# Autodesk Inventor assembly: CL4-400-GB
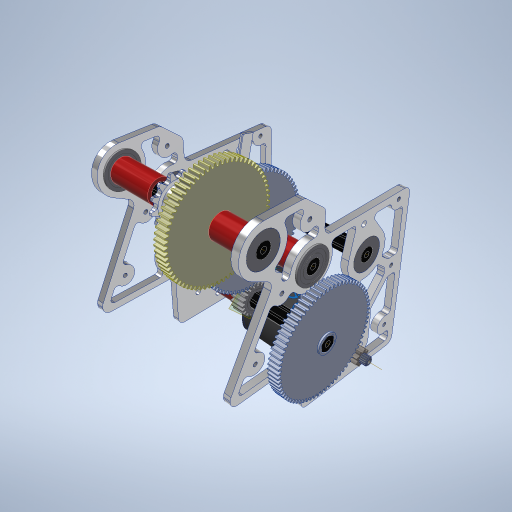
[picture p0: Inventor's stored thumbnail of the model, 512x512]
Saved by Autodesk Inventor 2023.4 (Build 274418000, 418)
## iProperties
Created: 2025-02-08
Part Number: CL4-400-GB
Document SubType Name: Assembly
Designer: slick
Mass: 1317.22 g
Surface Area: 2022.83 cm^2
Volume: 570.049 cm^3
Density: 2.31072 g/cm^3
Author: slick
## Documents named in this file (23)
- C:\Users\jmcintyr\Documents\GitHub\2025-ReefScape---CAD\Climber\CL4\CL4-400-GB.iam
- C:\Users\jmcintyr\Documents\GitHub\2025-ReefScape---CAD\Climber\CL4\CL4-016.ipt
- C:\Users\jmcintyr\Documents\GitHub\2025-ReefScape---CAD\COMMON PARTS\BEARINGS\0_500_ID_x_1_125_OD_x_0_313_WD_Flanged_Bearing_217-2731.ipt
- C:\Users\jmcintyr\Documents\GitHub\2025-ReefScape---CAD\COMMON PARTS\MOTORS\Kracken with Cover and Boards.iam
- C:\Users\jmcintyr\Documents\GitHub\2025-ReefScape---CAD\COMMON PARTS\GEARS\WCP-1006\WCP-1006.ipt
- C:\Users\jmcintyr\Documents\GitHub\2025-ReefScape---CAD\COMMON PARTS\GEARS\20dp .5 hex\72t_Aluminum_Spur_Gear_20_DP_1_2_Hex_Bore_217-3576.ipt
- C:\Users\jmcintyr\Documents\GitHub\2025-ReefScape---CAD\COMMON PARTS\GEARS\20dp .5 hex\20t_Aluminum_Spur_Gear_20_DP_1_2_Hex_Bore_217-2702.ipt
- C:\Users\jmcintyr\Documents\GitHub\2025-ReefScape---CAD\COMMON PARTS\GEARS\20dp .5 hex\68t_Aluminum_Spur_Gear_20_DP_1_2_Hex_Bore_217-5477.ipt
- C:\Users\jmcintyr\Documents\GitHub\2025-ReefScape---CAD\Climber\CL4\CL4-018.ipt
- C:\Users\jmcintyr\Documents\GitHub\2025-ReefScape---CAD\Climber\CL4\CL4-019.ipt
- C:\Users\jmcintyr\Documents\GitHub\2025-ReefScape---CAD\COMMON PARTS\BEARINGS\13_75mm_1_2_ThunderHex_ID_x_1_125_OD_x_0_313_WD_Flanged_Bearing_217-4006_MIR.ipt
- C:\Users\jmcintyr\Documents\GitHub\2025-ReefScape---CAD\Climber\CL4\CL4-020.ipt
- C:\Users\jmcintyr\Documents\GitHub\2025-ReefScape---CAD\COMMON PARTS\HUBS\WCP-1388.ipt
- C:\Users\jmcintyr\Documents\GitHub\2025-ReefScape---CAD\STEP files\5163A16_Ratcheting Combination Wrench stubby.ipt
- C:\Users\jmcintyr\Documents\GitHub\2025-ReefScape---CAD\Climber\CL4\CL4-024.ipt
- C:\Users\jmcintyr\Documents\GitHub\2025-ReefScape---CAD\Climber\CL4\CL4-025.ipt
- C:\Users\jmcintyr\Documents\GitHub\2025-ReefScape---CAD\Climber\Spacers\CL-S-001.ipt
- C:\Users\jmcintyr\Documents\GitHub\2025-ReefScape---CAD\Climber\Spacers\CL-S-002.ipt
- C:\Users\jmcintyr\Documents\GitHub\2025-ReefScape---CAD\Climber\Spacers\CL-S-003.ipt
- C:\Users\jmcintyr\Documents\GitHub\2025-ReefScape---CAD\Climber\Spacers\CL-S-005.ipt
- C:\Users\jmcintyr\Documents\GitHub\2025-ReefScape---CAD\Climber\Spacers\CL-S-007.ipt
- C:\Users\jmcintyr\Documents\GitHub\2025-ReefScape---CAD\COMMON PARTS\SPROCKETS\35\12t_Aluminum_Hub_Sprocket_35_Chain_1_2_Hex_Bore_217-2662.ipt
- C:\Users\jmcintyr\Documents\GitHub\2025-ReefScape---CAD\COMMON PARTS\MOTORS\X 60 MOTOR SPACER.ipt
## Components (36 placed, 22 different names)
1. CL4-016:1 — Mate:1, Mate:2, Mate:3, Mate:4, Symmetry:1, Mate:19, Mate:20, Insert:8, Insert:14, Insert:15, Insert:17, Insert:22
2. CL4-016:2 — Mate:1, Mate:2, Mate:3, Symmetry:1, Insert:11, Insert:12, Insert:13, Insert:16, Mate:34, Insert:18
3. 0_500_ID_x_1_125_OD_x_0_313_WD_Flanged_Bearing_217-2731:1 — Insert:12, Mate:26, Flush:6, Mate:53
4. 0_500_ID_x_1_125_OD_x_0_313_WD_Flanged_Bearing_217-2731:2 — Insert:13, Mate:23, Flush:4, Mate:44, Mate:58
5. 0_500_ID_x_1_125_OD_x_0_313_WD_Flanged_Bearing_217-2731:3 — Mate:12, Insert:11, Mate:24, Flush:5
6. 0_500_ID_x_1_125_OD_x_0_313_WD_Flanged_Bearing_217-2731:5 — Mate:14, Insert:14, Mate:28
7. 0_500_ID_x_1_125_OD_x_0_313_WD_Flanged_Bearing_217-2731:6 — Insert:8, Mate:46
8. Kracken with Cover and Boards:1 [sub-assembly] — Mate:4, Mate:6, Mate:7, Mate:19, Mate:59, Insert:21
9. WCP-1006:1 — Mate:6, Mate:7
10. 72t_Aluminum_Spur_Gear_20_DP_1_2_Hex_Bore_217-3576:1 — Mate:11, Mate:20, Mate:25, Mate:57
11. 20t_Aluminum_Spur_Gear_20_DP_1_2_Hex_Bore_217-2702:1 — Mate:11, Flush:1, Mate:52
12. 72t_Aluminum_Spur_Gear_20_DP_1_2_Hex_Bore_217-3576:2 — Mate:12, Flush:1, Mate:13, Mate:22, Mate:50
13. 20t_Aluminum_Spur_Gear_20_DP_1_2_Hex_Bore_217-2702:2 — Mate:13, Flush:2, Mate:22, Mate:47, Mate:51
14. 68t_Aluminum_Spur_Gear_20_DP_1_2_Hex_Bore_217-5477:1 — Mate:14, Flush:2, Mate:28, Mate:41, Mate:43
15. CL4-018:1 — Mate:23, Flush:4, Mate:40, Mate:42, Mate:45
16. CL4-019:1 — Mate:24, Flush:5
17. 13_75mm_1_2_ThunderHex_ID_x_1_125_OD_x_0_313_WD_Flanged_Bearing_217-4006_MIR:1 — Insert:15, Mate:25, Mate:56
18. CL4-020:1 — Mate:26, Flush:6
19. 0_500_ID_x_1_125_OD_x_0_313_WD_Flanged_Bearing_217-2731:7 — Insert:16, Mate:36
20. 0_500_ID_x_1_125_OD_x_0_313_WD_Flanged_Bearing_217-2731:8 — Insert:17, Mate:29, Flush:7
21. CL4-018:2 — Mate:29, Flush:7, Mate:32, Mate:33, Mate:35, Angle:1, Mate:39
22. WCP-1388:1 — Mate:30, Mate:31, Mate:34, Mate:37
23. WCP-1388:2 — Mate:30, Mate:31, Mate:32, Mate:33, Mate:37, Angle:1, Insert:19, Insert:20
24. 5163A16_Ratcheting Combination Wrench stubby:1 — Mate:35, Mate:36
25. CL4-024:1 — Insert:18
26. CL4-025:1 — Mate:38, Flush:8, Flush:9
27. CL4-025:2 — Mate:38, Flush:8, Flush:9, Mate:39, Insert:19, Insert:20
28. CL-S-001:1 — Mate:40, Mate:41
29. CL-S-002:1 — Mate:42, Mate:43
30. CL-S-003:1 — Mate:44, Mate:45
31. CL-S-001:2 — Mate:46, Mate:47
32. CL-S-005:1 — Mate:50, Mate:51
33. CL-S-005:2 — Mate:52, Mate:53
34. CL-S-007:1 — Mate:56, Mate:57
35. 12t_Aluminum_Hub_Sprocket_35_Chain_1_2_Hex_Bore_217-2662:1 — Mate:58
36. X 60 MOTOR SPACER:1 — Mate:59, Insert:21, Insert:22
## Relationships (69: Mate 45, Insert 13, Flush 9, Symmetry 1, Angle 1)
- Mate:1: CL4-016:1 ↔ CL4-016:2
- Mate:2: CL4-016:1 ↔ CL4-016:2
- Mate:3 (130.175 mm): CL4-016:1 ↔ CL4-016:2
- Mate:4: CL4-016:1 ↔ Kracken with Cover and Boards:1
- Mate:6: Kracken with Cover and Boards:1 ↔ WCP-1006:1
- Mate:7 (6.35 mm): Kracken with Cover and Boards:1 ↔ WCP-1006:1
- Mate:11: 72t_Aluminum_Spur_Gear_20_DP_1_2_Hex_Bore_217-3576:1 ↔ 20t_Aluminum_Spur_Gear_20_DP_1_2_Hex_Bore_217-2702:1
- Mate:12: 0_500_ID_x_1_125_OD_x_0_313_WD_Flanged_Bearing_217-2731:3 ↔ 72t_Aluminum_Spur_Gear_20_DP_1_2_Hex_Bore_217-3576:2
- Flush:1: 20t_Aluminum_Spur_Gear_20_DP_1_2_Hex_Bore_217-2702:1 ↔ 72t_Aluminum_Spur_Gear_20_DP_1_2_Hex_Bore_217-3576:2
- Mate:13: 72t_Aluminum_Spur_Gear_20_DP_1_2_Hex_Bore_217-3576:2 ↔ 20t_Aluminum_Spur_Gear_20_DP_1_2_Hex_Bore_217-2702:2
- Mate:14: 0_500_ID_x_1_125_OD_x_0_313_WD_Flanged_Bearing_217-2731:5 ↔ 68t_Aluminum_Spur_Gear_20_DP_1_2_Hex_Bore_217-5477:1
- Flush:2: 20t_Aluminum_Spur_Gear_20_DP_1_2_Hex_Bore_217-2702:2 ↔ 68t_Aluminum_Spur_Gear_20_DP_1_2_Hex_Bore_217-5477:1
- Symmetry:1: CL4-016:1 ↔ CL4-016:2
- Flush:3
- Mate:19 (6.35 mm): CL4-016:1 ↔ Kracken with Cover and Boards:1
- Mate:20 (3.175 mm): CL4-016:1 ↔ 72t_Aluminum_Spur_Gear_20_DP_1_2_Hex_Bore_217-3576:1
- Insert:8: CL4-016:1 ↔ 0_500_ID_x_1_125_OD_x_0_313_WD_Flanged_Bearing_217-2731:6
- Insert:11: CL4-016:2 ↔ 0_500_ID_x_1_125_OD_x_0_313_WD_Flanged_Bearing_217-2731:3
- Insert:12: CL4-016:2 ↔ 0_500_ID_x_1_125_OD_x_0_313_WD_Flanged_Bearing_217-2731:1
- Insert:13: CL4-016:2 ↔ 0_500_ID_x_1_125_OD_x_0_313_WD_Flanged_Bearing_217-2731:2
- Insert:14: CL4-016:1 ↔ 0_500_ID_x_1_125_OD_x_0_313_WD_Flanged_Bearing_217-2731:5
- Mate:22 (3.175 mm): 72t_Aluminum_Spur_Gear_20_DP_1_2_Hex_Bore_217-3576:2 ↔ 20t_Aluminum_Spur_Gear_20_DP_1_2_Hex_Bore_217-2702:2
- Mate:23: 0_500_ID_x_1_125_OD_x_0_313_WD_Flanged_Bearing_217-2731:2 ↔ CL4-018:1
- Flush:4: 0_500_ID_x_1_125_OD_x_0_313_WD_Flanged_Bearing_217-2731:2 ↔ CL4-018:1
- Mate:24: 0_500_ID_x_1_125_OD_x_0_313_WD_Flanged_Bearing_217-2731:3 ↔ CL4-019:1
- Flush:5: 0_500_ID_x_1_125_OD_x_0_313_WD_Flanged_Bearing_217-2731:3 ↔ CL4-019:1
- Insert:15: CL4-016:1 ↔ 13_75mm_1_2_ThunderHex_ID_x_1_125_OD_x_0_313_WD_Flanged_Bearing_217-4006_MIR:1
- Mate:25: 72t_Aluminum_Spur_Gear_20_DP_1_2_Hex_Bore_217-3576:1 ↔ 13_75mm_1_2_ThunderHex_ID_x_1_125_OD_x_0_313_WD_Flanged_Bearing_217-4006_MIR:1
- Mate:26: 0_500_ID_x_1_125_OD_x_0_313_WD_Flanged_Bearing_217-2731:1 ↔ CL4-020:1
- Flush:6: 0_500_ID_x_1_125_OD_x_0_313_WD_Flanged_Bearing_217-2731:1 ↔ CL4-020:1
- Mate:28 (28.575 mm): 0_500_ID_x_1_125_OD_x_0_313_WD_Flanged_Bearing_217-2731:5 ↔ 68t_Aluminum_Spur_Gear_20_DP_1_2_Hex_Bore_217-5477:1
- Insert:16: CL4-016:2 ↔ 0_500_ID_x_1_125_OD_x_0_313_WD_Flanged_Bearing_217-2731:7
- Insert:17: CL4-016:1 ↔ 0_500_ID_x_1_125_OD_x_0_313_WD_Flanged_Bearing_217-2731:8
- Mate:29: 0_500_ID_x_1_125_OD_x_0_313_WD_Flanged_Bearing_217-2731:8 ↔ CL4-018:2
- Flush:7: 0_500_ID_x_1_125_OD_x_0_313_WD_Flanged_Bearing_217-2731:8 ↔ CL4-018:2
- Mate:30: WCP-1388:1 ↔ WCP-1388:2
- Mate:31 (12.7 mm): WCP-1388:1 ↔ WCP-1388:2
- Mate:32: CL4-018:2 ↔ WCP-1388:2
- Mate:33: CL4-018:2 ↔ WCP-1388:2
- Mate:34 (44.45 mm): CL4-016:2 ↔ WCP-1388:1
- Mate:35: CL4-018:2 ↔ 5163A16_Ratcheting Combination Wrench stubby:1
- Mate:36: 0_500_ID_x_1_125_OD_x_0_313_WD_Flanged_Bearing_217-2731:7 ↔ 5163A16_Ratcheting Combination Wrench stubby:1
- Mate:37: WCP-1388:1 ↔ WCP-1388:2
- Angle:1 (0 deg): CL4-018:2 ↔ WCP-1388:2
- Insert:18: CL4-016:2 ↔ CL4-024:1
- Mate:38: CL4-025:1 ↔ CL4-025:2
- Flush:8: CL4-025:1 ↔ CL4-025:2
- Flush:9: CL4-025:1 ↔ CL4-025:2
- Mate:39: CL4-018:2 ↔ CL4-025:2
- Insert:19: WCP-1388:2 ↔ CL4-025:2
- Insert:20: WCP-1388:2 ↔ CL4-025:2
- Mate:40: CL4-018:1 ↔ CL-S-001:1
- Mate:41: 68t_Aluminum_Spur_Gear_20_DP_1_2_Hex_Bore_217-5477:1 ↔ CL-S-001:1
- Mate:42: CL4-018:1 ↔ CL-S-002:1
- Mate:43: 68t_Aluminum_Spur_Gear_20_DP_1_2_Hex_Bore_217-5477:1 ↔ CL-S-002:1
- Mate:44: 0_500_ID_x_1_125_OD_x_0_313_WD_Flanged_Bearing_217-2731:2 ↔ CL-S-003:1
- Mate:45: CL4-018:1 ↔ CL-S-003:1
- Mate:46: 0_500_ID_x_1_125_OD_x_0_313_WD_Flanged_Bearing_217-2731:6 ↔ CL-S-001:2
- Mate:47: 20t_Aluminum_Spur_Gear_20_DP_1_2_Hex_Bore_217-2702:2 ↔ CL-S-001:2
- Mate:50: 72t_Aluminum_Spur_Gear_20_DP_1_2_Hex_Bore_217-3576:2 ↔ CL-S-005:1
- Mate:51: 20t_Aluminum_Spur_Gear_20_DP_1_2_Hex_Bore_217-2702:2 ↔ CL-S-005:1
- Mate:52: 20t_Aluminum_Spur_Gear_20_DP_1_2_Hex_Bore_217-2702:1 ↔ CL-S-005:2
- Mate:53: 0_500_ID_x_1_125_OD_x_0_313_WD_Flanged_Bearing_217-2731:1 ↔ CL-S-005:2
- Mate:56: 13_75mm_1_2_ThunderHex_ID_x_1_125_OD_x_0_313_WD_Flanged_Bearing_217-4006_MIR:1 ↔ CL-S-007:1
- Mate:57: 72t_Aluminum_Spur_Gear_20_DP_1_2_Hex_Bore_217-3576:1 ↔ CL-S-007:1
- Mate:58: 0_500_ID_x_1_125_OD_x_0_313_WD_Flanged_Bearing_217-2731:2 ↔ 12t_Aluminum_Hub_Sprocket_35_Chain_1_2_Hex_Bore_217-2662:1
- Mate:59: Kracken with Cover and Boards:1 ↔ X 60 MOTOR SPACER:1
- Insert:21: Kracken with Cover and Boards:1 ↔ X 60 MOTOR SPACER:1
- Insert:22: CL4-016:1 ↔ X 60 MOTOR SPACER:1
